# Autodesk Inventor assembly: Montaje_Final
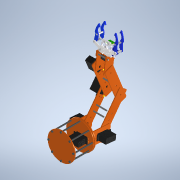
[picture p0: Inventor's stored thumbnail of the model, 180x180]
Saved by Autodesk Inventor 2021 (Build 250183000, 183)
## iProperties
Created: 2021-04-02
Part Number: Montaje_Final
Document SubType Name: Assembly
Designer: diego
Author: diego
## Documents named in this file (10)
- C:\Users\diego\Desktop\Diego\Utadeo 2021-1\Robotica Industrial\Corte 2\Solido planos\Montaje_Final.iam
- C:\Users\diego\Desktop\Diego\Utadeo 2021-1\Robotica Industrial\Corte 2\Solido planos\Base2.ipt
- C:\Users\diego\Desktop\Diego\Utadeo 2021-1\Robotica Industrial\Corte 2\Solido planos\7.ipt
- C:\Users\diego\Desktop\Diego\Utadeo 2021-1\Robotica Industrial\Corte 2\Solido planos\Extension2.ipt
- C:\Users\diego\Desktop\Diego\Utadeo 2021-1\Robotica Industrial\Corte 2\Solido planos\Servo.ipt
- C:\Users\diego\Desktop\Diego\Utadeo 2021-1\Robotica Industrial\Corte 2\Solido planos\Ensamblaje3.iam
- C:\Users\diego\Desktop\Diego\Utadeo 2021-1\Robotica Industrial\Corte 2\Solido planos\Ensamble.iam
- C:\Users\diego\Desktop\Diego\Utadeo 2021-1\Robotica Industrial\Corte 2\Solido planos\Ensamblaje4.iam
- C:\Users\diego\Desktop\Diego\Utadeo 2021-1\Robotica Industrial\Corte 2\Solido planos\Ensamblaje5.iam
- C:\Users\diego\Desktop\Diego\Utadeo 2021-1\Robotica Industrial\Corte 2\Gripper2\Autodesk Inventor\_Robotic Gripper Assembly.iam
## Components (10 placed, 9 different names)
1. Base2:1 — Coincidencia:1, Coincidencia:2, De rotación:4
2. Extension2:1 — Coincidencia:1, Coincidencia:2, Coincidencia:3
3. 7:1 — Coincidencia:3, De rotación:1, De rotación:2
4. Servo:1 — De rotación:1
5. Servo:2 — De rotación:2, De rotación:5
6. Ensamble:1 [sub-assembly] — De rotación:4
7. Ensamblaje3:1 [sub-assembly] — De rotación:5, De rotación:6, De rotación:7
8. Ensamblaje4:1 [sub-assembly] — De rotación:6, De rotación:7, De rotación:8
9. Ensamblaje5:1 [sub-assembly] — De rotación:8, Coincidencia:4
10. _Robotic Gripper Assembly:1 [sub-assembly] — Coincidencia:4
## Relationships (11: RevoluteJoint 7, Mate 4)
- Coincidencia:1 [Mate]: Base2:1 ↔ Extension2:1
- Coincidencia:2 [Mate]: Base2:1 ↔ Extension2:1
- Coincidencia:3 [Mate]: Extension2:1 ↔ 7:1
- De rotación:1 [RevoluteJoint] (3 mm): 7:1 ↔ Servo:1
- De rotación:2 [RevoluteJoint] (-3 mm): 7:1 ↔ Servo:2
- De rotación:4 [RevoluteJoint]: Base2:1 ↔ Ensamble:1
- De rotación:5 [RevoluteJoint] (-3 mm): Servo:2 ↔ Ensamblaje3:1
- De rotación:6 [RevoluteJoint] (-3 mm): Ensamblaje3:1 ↔ Ensamblaje4:1
- De rotación:7 [RevoluteJoint] (-3 mm): Ensamblaje3:1 ↔ Ensamblaje4:1
- De rotación:8 [RevoluteJoint]: Ensamblaje4:1 ↔ Ensamblaje5:1
- Coincidencia:4 [Mate]: Ensamblaje5:1 ↔ _Robotic Gripper Assembly:1
